# Autodesk Inventor assembly: fast_test_akkum
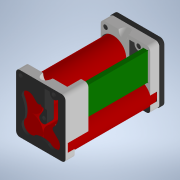
[picture p0: Inventor's stored thumbnail of the model, 180x180]
Saved by Autodesk Inventor 2022 (Build 260153000, 153)
## iProperties
Created: 2022-12-05
Part Number: fast_test_akkum
Document SubType Name: Assembly
Designer: akapu
Author: akapu
## Documents named in this file (6)
- C:\Users\akapu\OneDrive\Документы\maze bot\fast_test_akkum.iam
- C:\Users\akapu\OneDrive\Документы\maze bot\fast_test_akkum.ipt
- C:\Users\akapu\OneDrive\Документы\maze bot\test_18650.ipt
- C:\Users\akapu\OneDrive\Документы\maze bot\akkum_board2.ipt
- C:\Users\akapu\OneDrive\Документы\maze bot\fast_test_akkum_2.ipt
- C:\Users\akapu\OneDrive\Документы\maze bot\test_akkum_shelki.ipt
## Components (7 placed, 5 different names)
1. fast_test_akkum:1 — Rotational:1, Rotational:2, Rotational:3, Rotational:4, Flush:1
2. test_18650:1 — Rotational:1, Rotational:5
3. test_18650:2 — Rotational:2
4. test_18650:3 — Rotational:3, Mate:1
5. akkum_board2:1 — Rotational:4
6. fast_test_akkum_2:1 — Rotational:5, Mate:1
7. test_akkum_shelki:1 — Flush:1
## Relationships (7: RevoluteJoint 5, Mate 1, Flush 1)
- Rotational:1 [RevoluteJoint]: fast_test_akkum:1 ↔ test_18650:1
- Rotational:2 [RevoluteJoint]: fast_test_akkum:1 ↔ test_18650:2
- Rotational:3 [RevoluteJoint]: fast_test_akkum:1 ↔ test_18650:3
- Rotational:4 [RevoluteJoint]: fast_test_akkum:1 ↔ akkum_board2:1
- Rotational:5 [RevoluteJoint]: test_18650:1 ↔ fast_test_akkum_2:1
- Mate:1: test_18650:3 ↔ fast_test_akkum_2:1
- Flush:1: fast_test_akkum:1 ↔ test_akkum_shelki:1
